# Autodesk Inventor assembly: Microcontroller with VEXnet Microcontroller Upgrade Module
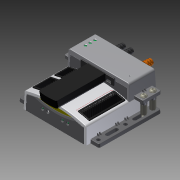
[picture p0: Inventor's stored thumbnail of the model, 180x180]
Saved by Autodesk Inventor 2015 SP1 (Build 190201100, 201)
## iProperties
Created: 2010-04-29
Part Number: Microcontroller with VEXnet Microcontroller Upgrade Module
Document SubType Name: Assembly
Designer: Jordan
Mass: 195.402 g
Surface Area: 1360.3 cm^2
Volume: 127.575 cm^3
Density: 1.53167 g/cm^3
Translation Standard: STEP AP214IS
FileName: Microcontroller with VEXnet Microcontroller Upgrade Module.iam
PreProcessor: SolidWorks 2009
PostProcessor: Build: 239, Release: 2011 RTM - Date: Wed 02/17/2010
Sent Units: inch
Uncertainty: 1e-05
Author: Jordan
## Documents named in this file (7)
- C:\Users\Jordan\Documents\Robotics\VEX\CAD\2015 BNS CAD Library (beta)\Logic\PIC Microcontroller V0.5 with VEXnet Upgrade Module.iam
- C:\Users\Jordan\Documents\Robotics\VEX\CAD\2015 BNS CAD Library (beta)\Structure\Screws & Nuts\Screw 8-32 x 0.500''.ipt
- C:\Users\Jordan\Documents\Robotics\VEX\CAD\2015 BNS CAD Library (beta)\Structure\Standoffs & Couplers\Standoff 0.50''.ipt
- C:\Users\Jordan\Documents\Robotics\VEX\CAD\2015 BNS CAD Library (beta)\Logic\Reference Parts\PIC Microcontroller V0.5 with VEXnet Upgrade Module\RX Controller.iam
- C:\Users\Jordan\Documents\Robotics\VEX\CAD\2015 BNS CAD Library (beta)\Logic\Reference Parts\VEXnet Microcontrollers\VEXnet USB Adapter Key.ipt
- C:\Users\Jordan\Documents\Robotics\VEX\CAD\2015 BNS CAD Library (beta)\Logic\Reference Parts\PIC Microcontroller V0.5 with VEXnet Upgrade Module\Reference Parts\RX Controller\Velcro Dot.ipt
- C:\Users\Jordan\Documents\Robotics\VEX\CAD\2015 BNS CAD Library (beta)\Logic\PIC Microcontroller V0.5.iam
## Components (17 placed, 6 different names)
1. Screw 8-32 x 0.500'':1 — Mate:11, Mate:12
2. Screw 8-32 x 0.500'':2 — Mate:21, Mate:22
3. Standoff 0.50'':1 — Mate:15, Mate:16, Mate:17, Mate:18
4. Screw 8-32 x 0.500'':3 — Mate:3, Mate:4
5. Standoff 0.50'':2 — Mate:13, Mate:14, Mate:23
6. Screw 8-32 x 0.500'':4 — Mate:9, Mate:10
7. Screw 8-32 x 0.500'':5 — Mate:1, Mate:2
8. Screw 8-32 x 0.500'':6 — Mate:19, Mate:20
9. Standoff 0.50'':3 — Mate:29, Mate:30
10. Standoff 0.50'':4 — Mate:27, Mate:28
11. RX Controller:1 [sub-assembly] — Mate:1, Mate:2, Mate:3, Mate:4, Mate:17, Mate:18, Mate:19, Mate:20, Mate:21, Mate:22, Mate:23, Mate:24, Mate:25, Mate:26, Mate:28, Mate:30
12. Screw 8-32 x 0.500'':7 — Mate:5, Mate:6
13. VEXnet USB Adapter Key:1 — Mate:24, Mate:25, Mate:26
14. Velcro Dot:1
15. Velcro Dot:2
16. Screw 8-32 x 0.500'':8 — Mate:7, Mate:8
17. PIC Microcontroller V0.5:1 [sub-assembly] — Mate:5, Mate:6, Mate:7, Mate:8, Mate:9, Mate:10, Mate:11, Mate:12, Mate:13, Mate:14, Mate:15, Mate:16, Mate:27, Mate:29
## Relationships (30: Mate 30)
- Mate:1: Screw 8-32 x 0.500'':5 ↔ RX Controller:1
- Mate:2: Screw 8-32 x 0.500'':5 ↔ RX Controller:1
- Mate:3: Screw 8-32 x 0.500'':3 ↔ RX Controller:1
- Mate:4: Screw 8-32 x 0.500'':3 ↔ RX Controller:1
- Mate:5: Screw 8-32 x 0.500'':7 ↔ PIC Microcontroller V0.5:1
- Mate:6: Screw 8-32 x 0.500'':7 ↔ PIC Microcontroller V0.5:1
- Mate:7: Screw 8-32 x 0.500'':8 ↔ PIC Microcontroller V0.5:1
- Mate:8: Screw 8-32 x 0.500'':8 ↔ PIC Microcontroller V0.5:1
- Mate:9: Screw 8-32 x 0.500'':4 ↔ PIC Microcontroller V0.5:1
- Mate:10: Screw 8-32 x 0.500'':4 ↔ PIC Microcontroller V0.5:1
- Mate:11: Screw 8-32 x 0.500'':1 ↔ PIC Microcontroller V0.5:1
- Mate:12: Screw 8-32 x 0.500'':1 ↔ PIC Microcontroller V0.5:1
- Mate:13: Standoff 0.50'':2 ↔ PIC Microcontroller V0.5:1
- Mate:14: Standoff 0.50'':2 ↔ PIC Microcontroller V0.5:1
- Mate:15: Standoff 0.50'':1 ↔ PIC Microcontroller V0.5:1
- Mate:16: Standoff 0.50'':1 ↔ PIC Microcontroller V0.5:1
- Mate:17: Standoff 0.50'':1 ↔ RX Controller:1
- Mate:18: Standoff 0.50'':1 ↔ RX Controller:1
- Mate:19: Screw 8-32 x 0.500'':6 ↔ RX Controller:1
- Mate:20: Screw 8-32 x 0.500'':6 ↔ RX Controller:1
- Mate:21: Screw 8-32 x 0.500'':2 ↔ RX Controller:1
- Mate:22: Screw 8-32 x 0.500'':2 ↔ RX Controller:1
- Mate:23: Standoff 0.50'':2 ↔ RX Controller:1
- Mate:24: RX Controller:1 ↔ VEXnet USB Adapter Key:1
- Mate:25: RX Controller:1 ↔ VEXnet USB Adapter Key:1
- Mate:26: RX Controller:1 ↔ VEXnet USB Adapter Key:1
- Mate:27: Standoff 0.50'':4 ↔ PIC Microcontroller V0.5:1
- Mate:28: Standoff 0.50'':4 ↔ RX Controller:1
- Mate:29: Standoff 0.50'':3 ↔ PIC Microcontroller V0.5:1
- Mate:30: Standoff 0.50'':3 ↔ RX Controller:1
